# Autodesk Inventor assembly: Assembly1
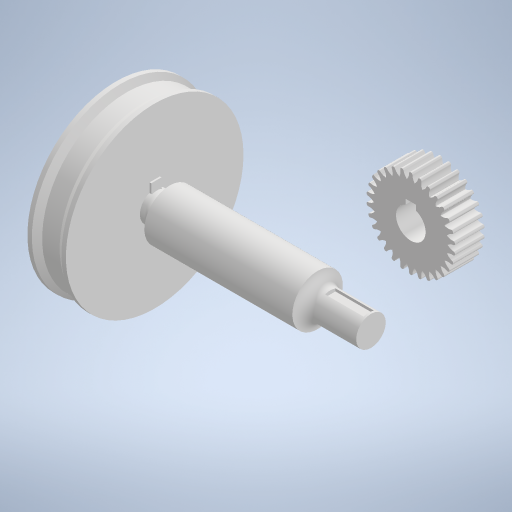
[picture p0: Inventor's stored thumbnail of the model, 512x512]
Saved by Autodesk Inventor 2024 (Build 280153000, 153)
## iProperties
Created: 2024-03-20
Part Number: Assembly1
Document SubType Name: Assembly
Designer: USUARIO
Author: USUARIO
## Documents named in this file (5)
- C:\Users\USUARIO\Documents\2024\UNIVERSIDAD\DINAMICA\LAB\Assembly1.iam
- C:\Users\USUARIO\Downloads\EJE_CUÑEROS.ipt
- C:\Users\USUARIO\Downloads\ENGRANE.ipt
- C:\Users\USUARIO\Downloads\POLEA.ipt
- C:\Users\USUARIO\Downloads\CUÑA.ipt
## Components (4 placed, 4 different names)
1. EJE_CUÑEROS:1 — Rotational:1, Flush:1, Mate:1, Rigid:1
2. ENGRANE:1
3. POLEA:1 — Rotational:1, Flush:1, Mate:1
4. CUÑA:1 — Rigid:1
## Relationships (4: RevoluteJoint 1, Flush 1, Mate 1, WeldJoint 1)
- Rotational:1 [RevoluteJoint]: EJE_CUÑEROS:1 ↔ POLEA:1
- Flush:1: EJE_CUÑEROS:1 ↔ POLEA:1
- Mate:1: EJE_CUÑEROS:1 ↔ POLEA:1
- Rigid:1 [WeldJoint]: EJE_CUÑEROS:1 ↔ CUÑA:1
